# Autodesk Inventor assembly: Front Left Wheel Hub Assemby
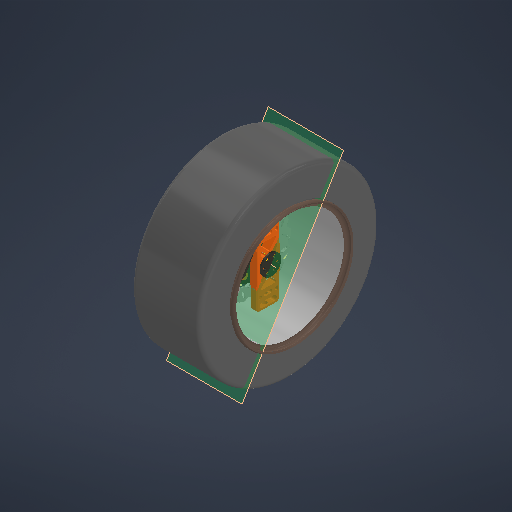
[picture p0: Inventor's stored thumbnail of the model, 512x512]
Saved by Autodesk Inventor 2026.1 (Build 301233000, 233)
## iProperties
Created: 2026-06-24
Part Number: Front Left Wheel Hub Assemby
Document SubType Name: Assembly
Designer: share
Author: share
## Documents named in this file (8)
- C:\Users\share\OneDrive\Documents\Personal Projects\GOGO Kart\CAD\GOGO_KART_FSAE\Suspension\Upright Assembly\Front Left Wheel Hub Assemby.iam
- C:\Users\share\OneDrive\Documents\Personal Projects\GOGO Kart\CAD\GOGO_KART_FSAE\Suspension\Upright Assembly\Front Upright.ipt
- C:\Users\share\OneDrive\Documents\Personal Projects\GOGO Kart\CAD\GOGO_KART_FSAE\Suspension\Upright Assembly\F3 Front Caliper Bracket.ipt
- C:\Users\share\OneDrive\Documents\Personal Projects\GOGO Kart\CAD\GOGO_KART_FSAE\Drivetrain\Rear_Wheel_Hub_Assembly.iam
- C:\Users\share\OneDrive\Documents\Personal Projects\GOGO Kart\CAD\GOGO_KART_FSAE\Suspension\Upright Assembly\Arashi Rear Brake Disc Rotors.ipt
- C:\Users\share\OneDrive\Documents\Personal Projects\GOGO Kart\CAD\GOGO_KART_FSAE\Suspension\Upright Assembly\2385K101_Angular Contact Single Row Ball Bearing.ipt
- C:\Users\share\OneDrive\Documents\Personal Projects\GOGO Kart\CAD\GOGO_KART_FSAE\Suspension\Upright Assembly\GrabCads\RimARTDesign2.ipt
- C:\Users\share\OneDrive\Documents\Personal Projects\GOGO Kart\CAD\GOGO_KART_FSAE\Suspension\Upright Assembly\GrabCads\20.5x7HoosierTire43162.ipt
## Components (8 placed, 7 different names)
1. Front Upright:1 — Flush:1, Flush:2, Flush:3, Mate:1, Insert:5, Insert:6
2. F3 Front Caliper Bracket:1 — Mate:2, Mate:3
3. Rear_Wheel_Hub_Assembly:1 [sub-assembly] — Mate:1, Insert:3, Insert:4, Insert:7, Insert:8, Insert:9
4. Arashi Rear Brake Disc Rotors:1 — Insert:3, Insert:4, Mate:3
5. 2385K101_Angular Contact Single Row Ball Bearing:1 — Insert:6, Insert:7
6. 2385K101_Angular Contact Single Row Ball Bearing:2 — Insert:5
7. RimARTDesign2:1 — Insert:8, Insert:9, Insert:10, Flush:4
8. 20.5x7HoosierTire43162:1 — Insert:10, Flush:4
## Relationships (15: Insert 8, Flush 4, Mate 3)
- Flush:1: Front Upright:1
- Flush:2: Front Upright:1
- Flush:3: Front Upright:1
- Mate:1: Front Upright:1 ↔ Rear_Wheel_Hub_Assembly:1
- Insert:3: Rear_Wheel_Hub_Assembly:1 ↔ Arashi Rear Brake Disc Rotors:1
- Insert:4: Rear_Wheel_Hub_Assembly:1 ↔ Arashi Rear Brake Disc Rotors:1
- Insert:5: Front Upright:1 ↔ 2385K101_Angular Contact Single Row Ball Bearing:2
- Insert:6: Front Upright:1 ↔ 2385K101_Angular Contact Single Row Ball Bearing:1
- Insert:7: Rear_Wheel_Hub_Assembly:1 ↔ 2385K101_Angular Contact Single Row Ball Bearing:1
- Mate:2: F3 Front Caliper Bracket:1
- Mate:3: F3 Front Caliper Bracket:1 ↔ Arashi Rear Brake Disc Rotors:1
- Insert:8: Rear_Wheel_Hub_Assembly:1 ↔ RimARTDesign2:1
- Insert:9: Rear_Wheel_Hub_Assembly:1 ↔ RimARTDesign2:1
- Insert:10: RimARTDesign2:1 ↔ 20.5x7HoosierTire43162:1
- Flush:4: RimARTDesign2:1 ↔ 20.5x7HoosierTire43162:1
